# Autodesk Inventor assembly: handle-base
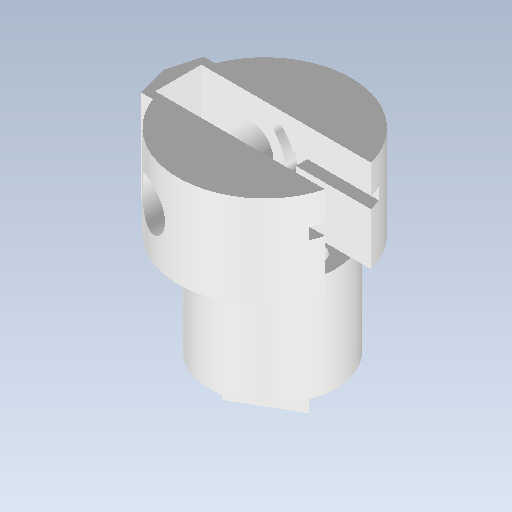
[picture p0: Inventor's stored thumbnail of the model, 512x512]
Saved by Autodesk Inventor 2021 (Build 250183000, 183)
## iProperties
Created: 2021-06-09
Part Number: handle-base
Document SubType Name: Assembly
Designer: teh18
Author: teh18
## Documents named in this file (3)
- C:\Users\teh18\OneDrive\BVE Controller\r68-bve-mascon\handle-base\handle-base.iam
- C:\Users\teh18\OneDrive\BVE Controller\r68-bve-mascon\handle-base\top.ipt
- C:\Users\teh18\OneDrive\BVE Controller\r68-bve-mascon\handle-base\bottom.ipt
## Components (2 placed, 2 different names)
1. top:1 — Mate:1, Mate:2
2. bottom:1 — Mate:1, Mate:2
## Relationships (2: Mate 2)
- Mate:1: top:1 ↔ bottom:1
- Mate:2: top:1 ↔ bottom:1
